# Autodesk Inventor assembly: CradleFlaskServo
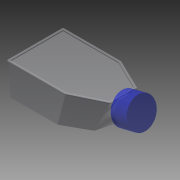
[picture p0: Inventor's stored thumbnail of the model, 180x180]
Saved by Autodesk Inventor 2014 SP1 (Build 180222100, 222)
## iProperties
Created: 2017-05-14
Part Number: CradleFlaskServo
Document SubType Name: Assembly
Designer: danielsikar
Author: danielsikar
## Documents named in this file (2)
- C:\Users\danielsikar\Documents\Inventor\FlaskCradle\assemblies\CradleFlaskServo.iam
- C:\Users\danielsikar\Documents\Inventor\FlaskCradle\parts\Flask.ipt
## Components (1 placed, 1 different names)
1. Flask:1 — Mate:1, Mate:2, Mate:3
## Relationships (3: Mate 3)
- Mate:1: Flask:1
- Mate:2: Flask:1
- Mate:3: Flask:1
